# Autodesk Inventor assembly: UBG-Stereokamera
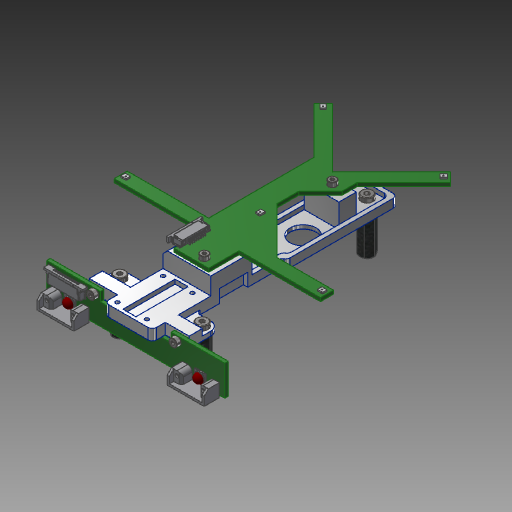
[picture p0: Inventor's stored thumbnail of the model, 512x512]
Saved by Autodesk Inventor 2019.4 (Build 234330000, 330)
## iProperties
Part Number: UBG-Stereokamera
Material: Generisch
Document SubType Name: Assembly
Designer: rYan
Mass: 59.45 g
Surface Area: 206.498 cm^2
Volume: 21.0082 cm^3
Density: 2.82984 g/cm^3
Author: rYan
## Documents named in this file (8)
- D:\TIGERsGIT\Hardware\mechanik\2020\Inventor\Robot\Electronics\UBG-Stereokamera.iam
- D:\TIGERsGIT\Hardware\mechanik\2020\Inventor\Robot\Electronics\Kameraplatte.ipt
- D:\TIGERsGIT\Hardware\mechanik\2019\Inventor\Kaufteile\Abstandsbolzen Typ A.ipt
- D:\TIGERsGIT\Hardware\mechanik\2020\Inventor\Inhaltscenter\de-DE\DIN 7984\DIN 7984 - M3 x 5.ipt
- D:\TIGERsGIT\Hardware\mechanik\2020\Inventor\Inhaltscenter\de-DE\ISO 4762(2)\ISO 4762 - M2 x 6ISO.ipt
- D:\TIGERsGIT\Hardware\mechanik\2020\Inventor\Purchased Parts\Abstandsbolzen Typ A M3 20mm SW6.ipt
- D:\TIGERsGIT\Hardware\mechanik\2020\Inventor\Robot\Electronics\MG-Eyeboard.iam
- D:\TIGERsGIT\Hardware\mechanik\2020\Inventor\Robot\Electronics\MG-Color Detect.iam
## Components (13 placed, 6 different names)
1. Kameraplatte:1 — Fluchtend:1, Fluchtend:2, Fluchtend:3, Einfügen:3, Einfügen:6, Einfügen:9, Einfügen:10, Einfügen:22, Einfügen:23, Einfügen:25, Einfügen:26, Passend:8
2. MG-Color Detect:1 [sub-assembly] — Passend:7, Passend:6, Einfügen:35, Einfügen:36, Passend:8
3. ISO 4762 M2 x 6:7 — Einfügen:35
4. ISO 4762 M2 x 6:8 — Einfügen:36
5. MG-Eyeboard:1 [sub-assembly] — Einfügen:25, Einfügen:26, Einfügen:33, Einfügen:34
6. ISO 4762 M2 x 6:5 — Einfügen:33
7. ISO 4762 M2 x 6:6 — Einfügen:34
8. Abstandsbolzen Typ A M3 20mm SW6:1 — Einfügen:3
9. Abstandsbolzen Typ A M3 20mm SW6:4 — Einfügen:6
10. Abstandsbolzen Typ A M3 20mm SW6:5 — Einfügen:22
11. DIN 7984 M3 x 5:1 — Einfügen:10
12. DIN 7984 M3 x 5:2 — Einfügen:9
13. DIN 7984 M3 x 5:3 — Einfügen:23
## Relationships (18: Insert 12, Flush 3, Mate 3)
- Fluchtend:1 [Flush]: Kameraplatte:1
- Fluchtend:2 [Flush]: Kameraplatte:1
- Fluchtend:3 [Flush]: Kameraplatte:1
- Einfügen:3 [Insert]: Kameraplatte:1 ↔ Abstandsbolzen Typ A M3 20mm SW6:1
- Einfügen:6 [Insert]: Kameraplatte:1 ↔ Abstandsbolzen Typ A M3 20mm SW6:4
- Einfügen:9 [Insert]: Kameraplatte:1 ↔ DIN 7984 M3 x 5:2
- Einfügen:10 [Insert]: Kameraplatte:1 ↔ DIN 7984 M3 x 5:1
- Einfügen:22 [Insert]: Kameraplatte:1 ↔ Abstandsbolzen Typ A M3 20mm SW6:5
- Einfügen:23 [Insert]: Kameraplatte:1 ↔ DIN 7984 M3 x 5:3
- Einfügen:25 [Insert]: Kameraplatte:1 ↔ MG-Eyeboard:1
- Einfügen:26 [Insert]: Kameraplatte:1 ↔ MG-Eyeboard:1
- Einfügen:33 [Insert]: MG-Eyeboard:1 ↔ ISO 4762 M2 x 6:5
- Einfügen:34 [Insert]: MG-Eyeboard:1 ↔ ISO 4762 M2 x 6:6
- Passend:7 [Mate]: MG-Color Detect:1
- Passend:6 [Mate]: MG-Color Detect:1
- Einfügen:35 [Insert]: MG-Color Detect:1 ↔ ISO 4762 M2 x 6:7
- Einfügen:36 [Insert]: MG-Color Detect:1 ↔ ISO 4762 M2 x 6:8
- Passend:8 [Mate]: Kameraplatte:1 ↔ MG-Color Detect:1
